# Autodesk Inventor assembly: ENCORDER_UNIT_RIGHT_KH
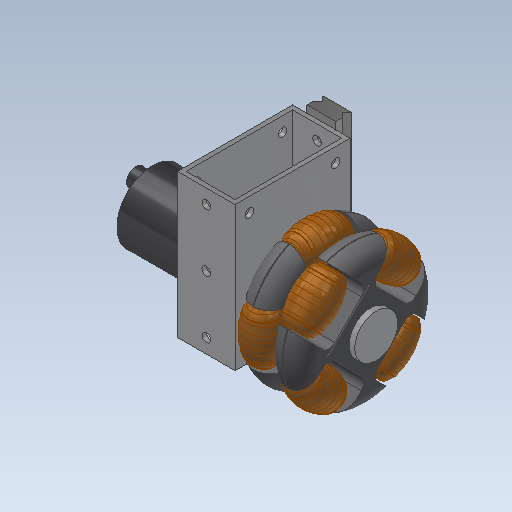
[picture p0: Inventor's stored thumbnail of the model, 512x512]
Saved by Autodesk Inventor 2020 (Build 240168000, 168)
## iProperties
Created: 2017-05-12
Part Number: ENCORDER_UNIT_RIGHT_KH
Material: 一般
Document SubType Name: Assembly
Designer: SHUICHI
Author: SHUICHI
## Documents named in this file (8)
- C:\Users\shun\Documents\Inventor\3wheel_omuni_2019\接地エンコーダーユニット\あ\ENCORDER_UNIT_RIGHT_KH.iam
- C:\Users\shun\Documents\Inventor\3wheel_omuni_2019\接地エンコーダーユニット\あ\K20X40X1P5_50_ENC_KH.ipt
- C:\Users\shun\Documents\Inventor\3wheel_omuni_2019\接地エンコーダーユニット\あ\ENCORDER_KH.ipt
- C:\Users\shun\Documents\Inventor\3wheel_omuni_2019\接地エンコーダーユニット\あ\BEAR_F13P8_12_8_ENC_KH.ipt
- C:\Users\shun\Documents\Inventor\3wheel_omuni_2019\接地エンコーダーユニット\あ\S14P9_45_ENC_KH.ipt
- C:\Users\shun\Documents\Inventor\3wheel_omuni_2019\接地エンコーダーユニット\あ\SPACER_14_8_2_ENC_KH.ipt
- C:\Users\shun\Documents\Inventor\3wheel_omuni_2019\接地エンコーダーユニット\あ\ROTACASTER_48_KH.iam
- C:\Users\shun\Documents\Inventor\3wheel_omuni_2019\接地エンコーダーユニット\あ\LINEAR_GUIDE_SSEB10_55_KH.ipt
## Components (7 placed, 7 different names)
1. K20X40X1P5_50_ENC_KH — 挿入:2, 挿入:5, メイト:1, 挿入:6, メイト:2
2. ENCORDER_KH — 挿入:5, メイト:1
3. BEAR_F13P8_12_8_ENC_KH — 挿入:2, 挿入:3
4. S14P9_45_ENC_KH — 挿入:1
5. SPACER_14_8_2_ENC_KH — 挿入:3, 挿入:4
6. ROTACASTER_48_KH [sub-assembly] — 挿入:1, 挿入:4
7. LINEAR_GUIDE_SSEB10_55_KH:1 — 挿入:6, メイト:2
## Relationships (8: Insert 6, Mate 2)
- 挿入:1 [Insert]: S14P9_45_ENC_KH ↔ ROTACASTER_48_KH
- 挿入:2 [Insert]: K20X40X1P5_50_ENC_KH ↔ BEAR_F13P8_12_8_ENC_KH
- 挿入:3 [Insert]: BEAR_F13P8_12_8_ENC_KH ↔ SPACER_14_8_2_ENC_KH
- 挿入:4 [Insert]: SPACER_14_8_2_ENC_KH ↔ ROTACASTER_48_KH
- 挿入:5 [Insert]: K20X40X1P5_50_ENC_KH ↔ ENCORDER_KH
- メイト:1 [Mate]: K20X40X1P5_50_ENC_KH ↔ ENCORDER_KH
- 挿入:6 [Insert]: K20X40X1P5_50_ENC_KH ↔ LINEAR_GUIDE_SSEB10_55_KH:1
- メイト:2 [Mate]: K20X40X1P5_50_ENC_KH ↔ LINEAR_GUIDE_SSEB10_55_KH:1
